# Autodesk Inventor assembly: Celda ensamblaje
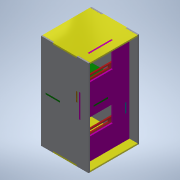
[picture p0: Inventor's stored thumbnail of the model, 180x180]
Saved by Autodesk Inventor 2020 (Build 240168000, 168)
## iProperties
Created: 2020-03-11
Part Number: Celda ensamblaje
Material: Genérico
Document SubType Name: Assembly
Designer: joser
Author: joser
## Documents named in this file (12)
- C:\Users\joser\OneDrive\Documentos\UVG\2020\Digital 2\Proyecto\Maqueta\Celda ensamblaje.iam
- C:\Users\joser\OneDrive\Documentos\UVG\2020\Digital 2\Proyecto\Maqueta\Celda Piso.ipt
- C:\Users\joser\OneDrive\Documentos\UVG\2020\Digital 2\Proyecto\Maqueta\Celda lateral.ipt
- C:\Users\joser\OneDrive\Documentos\UVG\2020\Digital 2\Proyecto\Maqueta\Celda celdas.ipt
- C:\Users\joser\OneDrive\Documentos\UVG\2020\Digital 2\Proyecto\Maqueta\Celda puertas.ipt
- C:\Users\joser\OneDrive\Documentos\UVG\2020\Digital 2\Proyecto\Maqueta\Celda pared divisora.ipt
- C:\Users\joser\OneDrive\Documentos\UVG\2020\Digital 2\Proyecto\Maqueta\celda base cremallera.ipt
- C:\Users\joser\OneDrive\Documentos\UVG\2020\Digital 2\Proyecto\Maqueta\Celda pared cremallera.ipt
- C:\Users\joser\OneDrive\Documentos\UVG\2020\Digital 2\Proyecto\Maqueta\Celda sos deslizador.ipt
- C:\Users\joser\OneDrive\Documentos\UVG\2020\Digital 2\Proyecto\Maqueta\Celda sos desli.ipt
- C:\Users\joser\OneDrive\Documentos\UVG\2020\Digital 2\Proyecto\Maqueta\Celda techo.ipt
- C:\Users\joser\OneDrive\Documentos\UVG\2020\Digital 2\Proyecto\Maqueta\Celda riel.ipt
## Components (12 placed, 11 different names)
1. Celda Piso:1 — Coincidencia:1, Coincidencia:2, Coincidencia:3, Coincidencia:4, Coincidencia:5, Coincidencia:6, Coincidencia:10, Coincidencia:14, Coincidencia:20, Coincidencia:33, Coincidencia:34, Coincidencia:35
2. Celda lateral:1 — Coincidencia:1, Coincidencia:2, Coincidencia:3, Coincidencia:11, Coincidencia:12
3. Celda lateral:2 — Coincidencia:4, Coincidencia:5, Coincidencia:6, Coincidencia:31, Coincidencia:32
4. Celda celdas:1 — Coincidencia:10, Coincidencia:11, Coincidencia:12, Coincidencia:13, Coincidencia:15, Coincidencia:19, Nivelación:1, Coincidencia:24, Coincidencia:25, Coincidencia:26
5. Celda puertas:1 — Coincidencia:16, Coincidencia:17, Coincidencia:18, Coincidencia:19, Coincidencia:20, Nivelación:1
6. Celda pared divisora:1 — Coincidencia:13, Coincidencia:14, Coincidencia:15, Coincidencia:30
7. celda base cremallera:1 — Coincidencia:16, Coincidencia:17, Coincidencia:18, Coincidencia:21, Coincidencia:22, Coincidencia:23
8. Celda pared cremallera:1 — Coincidencia:21, Coincidencia:22, Coincidencia:23
9. Celda sos deslizador:1 — Coincidencia:24, Coincidencia:25, Coincidencia:26, Coincidencia:27, Coincidencia:28, Coincidencia:29
10. Celda sos desli:1 — Coincidencia:27, Coincidencia:28, Coincidencia:29
11. Celda techo:1 — Coincidencia:30, Coincidencia:31, Coincidencia:32
12. Celda riel:1 — Coincidencia:33, Coincidencia:34, Coincidencia:35
## Relationships (33: Mate 32, Flush 1)
- Coincidencia:1 [Mate]: Celda Piso:1 ↔ Celda lateral:1
- Coincidencia:2 [Mate]: Celda Piso:1 ↔ Celda lateral:1
- Coincidencia:3 [Mate]: Celda Piso:1 ↔ Celda lateral:1
- Coincidencia:4 [Mate]: Celda Piso:1 ↔ Celda lateral:2
- Coincidencia:5 [Mate]: Celda Piso:1 ↔ Celda lateral:2
- Coincidencia:6 [Mate]: Celda Piso:1 ↔ Celda lateral:2
- Coincidencia:10 [Mate]: Celda Piso:1 ↔ Celda celdas:1
- Coincidencia:11 [Mate]: Celda lateral:1 ↔ Celda celdas:1
- Coincidencia:12 [Mate]: Celda lateral:1 ↔ Celda celdas:1
- Coincidencia:13 [Mate]: Celda celdas:1 ↔ Celda pared divisora:1
- Coincidencia:14 [Mate]: Celda Piso:1 ↔ Celda pared divisora:1
- Coincidencia:15 [Mate]: Celda celdas:1 ↔ Celda pared divisora:1
- Coincidencia:16 [Mate]: Celda puertas:1 ↔ celda base cremallera:1
- Coincidencia:17 [Mate]: Celda puertas:1 ↔ celda base cremallera:1
- Coincidencia:18 [Mate]: Celda puertas:1 ↔ celda base cremallera:1
- Coincidencia:19 [Mate]: Celda celdas:1 ↔ Celda puertas:1
- Coincidencia:20 [Mate]: Celda Piso:1 ↔ Celda puertas:1
- Nivelación:1 [Flush]: Celda celdas:1 ↔ Celda puertas:1
- Coincidencia:21 [Mate]: celda base cremallera:1 ↔ Celda pared cremallera:1
- Coincidencia:22 [Mate]: celda base cremallera:1 ↔ Celda pared cremallera:1
- Coincidencia:23 [Mate]: celda base cremallera:1 ↔ Celda pared cremallera:1
- Coincidencia:24 [Mate]: Celda celdas:1 ↔ Celda sos deslizador:1
- Coincidencia:25 [Mate]: Celda celdas:1 ↔ Celda sos deslizador:1
- Coincidencia:26 [Mate]: Celda celdas:1 ↔ Celda sos deslizador:1
- Coincidencia:27 [Mate]: Celda sos deslizador:1 ↔ Celda sos desli:1
- Coincidencia:28 [Mate]: Celda sos deslizador:1 ↔ Celda sos desli:1
- Coincidencia:29 [Mate]: Celda sos deslizador:1 ↔ Celda sos desli:1
- Coincidencia:30 [Mate]: Celda pared divisora:1 ↔ Celda techo:1
- Coincidencia:31 [Mate]: Celda lateral:2 ↔ Celda techo:1
- Coincidencia:32 [Mate]: Celda lateral:2 ↔ Celda techo:1
- Coincidencia:33 [Mate]: Celda Piso:1 ↔ Celda riel:1
- Coincidencia:34 [Mate]: Celda Piso:1 ↔ Celda riel:1
- Coincidencia:35 [Mate]: Celda Piso:1 ↔ Celda riel:1
